# Autodesk Inventor assembly: robotassembly1
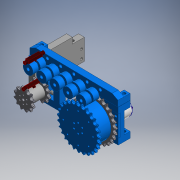
[picture p0: Inventor's stored thumbnail of the model, 180x180]
Saved by Autodesk Inventor 2016 (Build 200138000, 138)
## iProperties
Created: 2016-05-14
Part Number: robotassembly1
Document SubType Name: Assembly
Designer: hesaon
Author: hesaon
## Documents named in this file (16)
- C:\Users\hesaon\Documents\Killer-Bot-2016\AutodeskWorkspace\robotassembly1.iam
- C:\Users\hesaon\Documents\Killer-Bot-2016\AutodeskWorkspace\motorHolder57mmVer2.ipt
- C:\Users\hesaon\Documents\Killer-Bot-2016\AutodeskWorkspace\37D mm metal gearmotor.ipt
- C:\Users\hesaon\Documents\Killer-Bot-2016\AutodeskWorkspace\mountingHub6mm.ipt
- C:\Users\hesaon\Documents\Killer-Bot-2016\AutodeskWorkspace\sprocketsHolder.ipt
- C:\Users\hesaon\Documents\Killer-Bot-2016\AutodeskWorkspace\BigSprocket2.ipt
- C:\Users\hesaon\Documents\Killer-Bot-2016\AutodeskWorkspace\tracks_center.ipt
- C:\Users\hesaon\Documents\Killer-Bot-2016\AutodeskWorkspace\outerBigSprocket2.ipt
- C:\Users\hesaon\Documents\Killer-Bot-2016\AutodeskWorkspace\framesideRight.ipt
- C:\Users\hesaon\Documents\Killer-Bot-2016\AutodeskWorkspace\smallSprocketHolder.ipt
- C:\Users\hesaon\Documents\Killer-Bot-2016\AutodeskWorkspace\smallSprocket2.ipt
- C:\Users\hesaon\Documents\Killer-Bot-2016\AutodeskWorkspace\frameBack.ipt
- C:\Users\hesaon\Documents\Killer-Bot-2016\AutodeskWorkspace\pin5x60.ipt
- C:\Users\hesaon\Documents\Killer-Bot-2016\AutodeskWorkspace\smallSprocketFixture.ipt
- C:\Users\hesaon\Documents\Killer-Bot-2016\AutodeskWorkspace\roller.ipt
- C:\Users\hesaon\Documents\Killer-Bot-2016\AutodeskWorkspace\frameBottomRight.ipt
## Components (22 placed, 14 different names)
1. motorHolder57mmVer2:1 — Insert:1, Insert:2, Flush:2, Mate:5, Mate:6
2. 37D mm metal gearmotor:1 — Insert:1, Insert:2, Insert:3
3. mountingHub6mm:1 — Insert:3, Insert:9, Insert:10
4. sprocketsHolder:2 — Insert:7, Insert:8, Mate:1, Mate:2, Mate:3, Mate:4
5. Roller Chain Sprocket1:2 — Insert:7, Insert:8
6. Outer big sprocket:1 — Mate:1, Mate:2, Mate:3, Mate:4, Insert:9, Insert:10
7. framesideRight:1 — Flush:1, Insert:27, Insert:28, Flush:2, Mate:5, Insert:30, Mate:6
8. smallSprocketHolder:1 — Insert:13, Insert:14, Insert:15, Insert:16
9. Roller Chain Sprocket1:3 — Insert:13, Insert:14
10. Roller Chain Sprocket1:4 — Insert:15, Insert:16, Insert:17, Insert:26
11. tracks_center:2 — Insert:17
12. frameBack:1 — Flush:1, Cylindrical:1, Cylindrical:2
13. pin5x60:1 — Cylindrical:2, Cylindrical:3, Insert:27
14. pin5x60:2 — Insert:28
15. smallSprocketFixture:1 — Cylindrical:1, Cylindrical:3, Insert:26
16. roller:2 — Tangent:1, Flush:3, Flush:4, Insert:36
17. roller:3 — Insert:35
18. roller:4 — Insert:34
19. roller:5 — Insert:33
20. roller:6 — Insert:32
21. frameBottomRight:1 — Insert:30, Insert:32, Insert:33, Insert:34, Insert:35, Insert:36
22. tracks_center:3 — Tangent:1, Flush:3, Flush:4
## Relationships (35: Insert 21, Mate 6, Flush 4, CylindricalJoint 3, Tangent 1)
- Insert:1: motorHolder57mmVer2:1 ↔ 37D mm metal gearmotor:1
- Insert:2: motorHolder57mmVer2:1 ↔ 37D mm metal gearmotor:1
- Insert:3: 37D mm metal gearmotor:1 ↔ mountingHub6mm:1
- Insert:7: sprocketsHolder:2 ↔ Roller Chain Sprocket1:2
- Insert:8: sprocketsHolder:2 ↔ Roller Chain Sprocket1:2
- Mate:1: sprocketsHolder:2 ↔ Outer big sprocket:1
- Mate:2: sprocketsHolder:2 ↔ Outer big sprocket:1
- Mate:3: sprocketsHolder:2 ↔ Outer big sprocket:1
- Mate:4: sprocketsHolder:2 ↔ Outer big sprocket:1
- Insert:9: mountingHub6mm:1 ↔ Outer big sprocket:1
- Insert:10: mountingHub6mm:1 ↔ Outer big sprocket:1
- Insert:13: smallSprocketHolder:1 ↔ Roller Chain Sprocket1:3
- Insert:14: smallSprocketHolder:1 ↔ Roller Chain Sprocket1:3
- Insert:15: smallSprocketHolder:1 ↔ Roller Chain Sprocket1:4
- Insert:16: smallSprocketHolder:1 ↔ Roller Chain Sprocket1:4
- Insert:17: Roller Chain Sprocket1:4 ↔ tracks_center:2
- Flush:1: framesideRight:1 ↔ frameBack:1
- Cylindrical:1: frameBack:1 ↔ smallSprocketFixture:1
- Cylindrical:2: frameBack:1 ↔ pin5x60:1
- Cylindrical:3: pin5x60:1 ↔ smallSprocketFixture:1
- Insert:26 (6.5 mm): Roller Chain Sprocket1:4 ↔ smallSprocketFixture:1
- Insert:27: framesideRight:1 ↔ pin5x60:1
- Insert:28: framesideRight:1 ↔ pin5x60:2
- Flush:2: motorHolder57mmVer2:1 ↔ framesideRight:1
- Mate:5: motorHolder57mmVer2:1 ↔ framesideRight:1
- Tangent:1: roller:2 ↔ tracks_center:3
- Flush:3: roller:2 ↔ tracks_center:3
- Flush:4: roller:2 ↔ tracks_center:3
- Insert:30: framesideRight:1 ↔ frameBottomRight:1
- Insert:32 (12.16 mm): roller:6 ↔ frameBottomRight:1
- Insert:33 (12.16 mm): roller:5 ↔ frameBottomRight:1
- Insert:34 (12.16 mm): roller:4 ↔ frameBottomRight:1
- Insert:35 (12.16 mm): roller:3 ↔ frameBottomRight:1
- Insert:36 (12.16 mm): roller:2 ↔ frameBottomRight:1
- Mate:6: motorHolder57mmVer2:1 ↔ framesideRight:1
